# Autodesk Inventor assembly: CP96SDB40-160-M9PM(160_0_0)
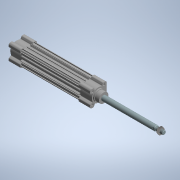
[picture p0: Inventor's stored thumbnail of the model, 180x180]
Saved by Autodesk Inventor 2021 (Build 250183000, 183)
## iProperties
Category: PARTsolutions
Company: SMC
Part Number: CP96SDB40-160-M9PM(160_0_0)
Catalog Web Link: www.cadenas.de
Description: CP96S/CP96SD-ISO Cylinder:Standard Double Acting,Single/Double Rod
Vendor: SMC
Document SubType Name: Assembly
Designer: partserver
Manufacturer: SMC
Mass: 418.331 g
Surface Area: 1384.59 cm^2
Volume: 418.331 cm^3
Density: 1 g/cm^3
PSOL_IDENT_0: {$CADENAS_DATA\23d-libs\smc_jp\actuator\standard_air_cylinder\cp96_c96\cp96_asmtab.prj},286 {VTYP=3D
PSOL_IDENT_1: },{STYP=ASSTAB},{NB=CP96SDB40-160-M9PM(160_0_0)},{LINA=CP96SDB40-160-M9PM},{NN=CP96S/CP96SD},{DATE=1
PSOL_IDENT_2: 8.06.2021 10:30:56},{GEOMDATE=24.12.2018 05:26:10},{VERSION=},{LINEID=20},{WBVAR=MAGNET,AUTOSWITCH,L
PSOL_IDENT_3: EAD,NUMBER,STROKE,POS,ROD,BOOT,STOP,ATEX,OMSC,THREAD},{WBNUMERIC=STROKE,POS}  {NB=CP96SDB40-160-M9PM
PSOL_IDENT_4: (160_0_0)},{LINA=CP96SDB40-160-M9PM},{KT=DUMMY},{BORE=40},{MOUNT=(B) Basic},{MOUNTX=B},{MAGNET=D},{A
PSOL_IDENT_5: UTOSWITCH=-M9P},{AUTOSWITCHX='','(-) Without autoswitch','-M9N','M9N','-M9P','M9P','-M9B','M9B','-M9
PSOL_IDENT_6: NW','M9NW','-M9PW','M9PW','-M9BW','M9BW','-M9NA','M9NA','-M9PA','M9PA','-M9BA','M9BA','-A96','A96','
PSOL_IDENT_7: -A93','A93','-A90','A90'},{SWITCH=B},{LEAD=M},{LEADX='','(-) 0.5 m','M','(M) 1 m','L','(L) 3 m','Z','
PSOL_IDENT_8: (Z) 5 m'},{NUMBER=},{NUMBERX='', '(-) 2 pcs', 'S', '(S) 1 pc'},{STROKE=160},{STDSTROKE=25,50,80,100,
PSOL_IDENT_9: 125,160,200,250,320,400,500},{STROKEX=25,50,80,100,125,160,200,250,320,400,500},{SMINX=15},{SMAX=200
PSOL_IDENT_10: 0},{SMAXX=2000},{POS=160},{ROD=},{RODX='','(-) Single rod','W','(W) Double rod'},{BOOT=},{BOOTX='','
PSOL_IDENT_11: (-) Without boot','J','(J) Nylon tarpaulin (one end)','K','(K) Heat resistant tarpaulin (one end)'},
PSOL_IDENT_12: {STOP=0},{STOPX='0','Standard stroke','1','Manufacturable stroke'},{COM=-},{ATEX=},{ATEXX='','N/A'},
PSOL_IDENT_13: {OMSC=},{OMSCX='','(-) Without order','-XC4','(-XC4) With heavy duty scraper','-XC7','(-XC7) Tie-rod
PSOL_IDENT_14: , cushion valve, tie-rod nut, etc. Made of stainless steel','-XC18','(-XC18) Port thread type NPT','
PSOL_IDENT_15: -XC22','(-XC22) Fluororubber seals','-XC35','(-XC35) With coil scraper','-XC68','(-XC68) Made of sta
PSOL_IDENT_16: inless steel (With hard chrome plated piston rod)'},{THREAD=0},{ORDER=CP96SDB40-160-M9PM},{A=24},{B=
PSOL_IDENT_17: 35},{D=16},{EE=G 1/4},{PL=14.0},{RT=M6x1},{L12=6.5},{KK=M12x1.25},{SW=13},{G=37.5},{BG=16},{L8=105},
PSOL_IDENT_18: {VD=4},{VA=4},{WA=5.0},{WB=9.0},{WH=30},{ZZ=163},{ZY=213},{E=54},{R=38.0},{L2=17},{L9=4},{H=54},{E1=
PSOL_IDENT_19: 55},{TR=36},{AH=36},{AO=11},{AT=4.5},{AB=10.0},{SA=161},{XA=163},{TM=63},{TL=16},{TD=16},{UW=58},{L1=
PSOL_IDENT_20: 22},{XV=82.5},{Z=106.5},{RF=36},{TF=72},{FB=9},{E2=55},{UF=90},{W=20},{MF=10},{ZF=145},{UB=52},{CB=2
PSOL_IDENT_21: 8},{EW=28-0.2/-0.6},{CD=12},{L=15},{MR=12.0},{XD=160},{EB=75},{A1=10.5},{A2=6.5},{B1=8.0},{B2=4.0},{
PSOL_IDENT_22: AA=10.5},{BB=8.0},{PPATH=cp96/assembly/cp96_asmsbl.prj},{MODEL=CP96SDB40-160-M9PM},{NENN=CP96SB40}
NB: CP96SDB40-160-M9PM(160_0_0)
NN: CP96S/CP96SD
NT: ISO Cylinder:Standard Double Acting,Single/Double Rod
NBSYN: $ORDER.($POS._$STOP._$THREAD.)
LINA: CP96SDB40-160-M9PM
CATALOG: SMC (JP
ROWDESC: CP96SB40
BORE: 40
MOUNT: (B) Basic
MAGNET: (D) With magnet
AUTOSWITCH: M9P Solid state-General-Grommet-Indicator light:Yes-3 wire(PNP)-In line
LEAD: (M) 1 m
NUMBER: (-) 2 pcs
STROKE: 160
POS: 160
ROD: (-) Single rod
BOOT: (-) Without boot
STOP: Standard stroke
COM: -
ATEX: N/A
OMSC: (-) Without order
THREAD: on
SUPPLIER: SMC
ARTICLENO: CP96SDB40-160-M9PM(160_0_0)
BOMINFO: CP96SDB40-160-M9PM
CREATOR: CADENAS GmbH
Title: CP96SDB40-160-M9PM
Author: Cadenas PARTsolutions
Comments: ISO Cylinder:Standard Double Acting,Single/Double Rod
## Documents named in this file (5)
- C:\Users\Nelson\Github\Proyecto_APM\Inventor_Corte\AIS2021\CP96SDB40-160-M9PM(160_0_0).iam
- C:\Users\Nelson\Github\Proyecto_APM\Inventor_Corte\AIS2021\CP96S40-160(0)_BODY.ipt
- C:\Users\Nelson\Github\Proyecto_APM\Inventor_Corte\AIS2021\CP96-M9P_SW.ipt
- C:\Users\Nelson\Github\Proyecto_APM\Inventor_Corte\AIS2021\CP96S40-160_ROD.ipt
- C:\Users\Nelson\Github\Proyecto_APM\Inventor_Corte\AIS2021\C96S40_NUT.ipt
## Components (5 placed, 4 different names)
1. CP96S40-160(0)_BODY:1 — Flush:1, Mate:1, Flush:2, Mate:2
2. CP96-M9P_SW:1 — Flush:1, Mate:1, Flush:3
3. CP96S40-160_ROD:1 — Flush:3, Flush:4
4. C96S40_NUT:1
5. CP96-M9P_SW:2 — Flush:2, Mate:2, Flush:4
## Relationships (6: Flush 4, Mate 2)
- Flush:1: CP96S40-160(0)_BODY:1 ↔ CP96-M9P_SW:1
- Mate:1 (0.1 mm): CP96S40-160(0)_BODY:1 ↔ CP96-M9P_SW:1
- Flush:2: CP96S40-160(0)_BODY:1 ↔ CP96-M9P_SW:2
- Mate:2 (0.1 mm): CP96S40-160(0)_BODY:1 ↔ CP96-M9P_SW:2
- Flush:3 (-2 mm): CP96-M9P_SW:1 ↔ CP96S40-160_ROD:1
- Flush:4 (162 mm): CP96S40-160_ROD:1 ↔ CP96-M9P_SW:2
